# Autodesk Inventor assembly: 2 Tall C-Channel Mount
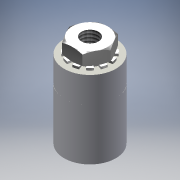
[picture p0: Inventor's stored thumbnail of the model, 180x180]
Saved by Autodesk Inventor 2019 (Build 230136000, 136)
## iProperties
Created: 2019-04-09
Part Number: 2 Tall C-Channel Mount
Document SubType Name: Assembly
Designer: thinkpad
Author: thinkpad
## Documents named in this file (4)
- F:\VEX Inventor Library\VEX Parts Library 2016\Imperial\Motion\2 Tall C-Channel Mount.iam
- F:\VEX Inventor Library\VEX Parts Library 2016\Imperial\Structure\Nut 8-32 Keps.ipt
- F:\VEX Inventor Library\VEX Parts Library 2016\Imperial\Motion\Nylon Spacer 0.5 inch.ipt
- F:\VEX Inventor Library\VEX Parts Library 2016\Imperial\Motion\Nylon Spacer 0.25 inch.ipt
## Components (3 placed, 3 different names)
1. Nut 8-32 Keps:1 — Mate:3, Mate:4
2. Nylon Spacer 0.5 inch:1 — Mate:1, Mate:2
3. Nylon Spacer 0.25 inch:1 — Mate:1, Mate:2, Mate:3, Mate:4
## Relationships (4: Mate 4)
- Mate:1: Nylon Spacer 0.5 inch:1 ↔ Nylon Spacer 0.25 inch:1
- Mate:2: Nylon Spacer 0.5 inch:1 ↔ Nylon Spacer 0.25 inch:1
- Mate:3: Nut 8-32 Keps:1 ↔ Nylon Spacer 0.25 inch:1
- Mate:4: Nut 8-32 Keps:1 ↔ Nylon Spacer 0.25 inch:1
